# Autodesk Inventor assembly: USE THIS FOR 2018 Practice Drivebase Assembly
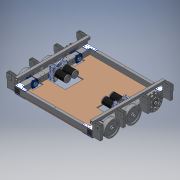
[picture p0: Inventor's stored thumbnail of the model, 180x180]
Saved by Autodesk Inventor 2019 (Build 230136000, 136)
## iProperties
Created: 2018-12-20
Part Number: USE THIS FOR 2018 Practice Drivebase Assembly
Document SubType Name: Assembly
Designer: Tiberus
Sending System: Autodesk Inventor 2018
Preprocessor: ST-DEVELOPER v16.13
Title: C:\Users\maste\OneDrive\Documents\GitHub\2019CAD\USE THIS FOR 2018 Practice Drivebase Assembly.stp
Author: maste
## Documents named in this file (6)
- C:\Users\Tiberus\Documents\Inventor\Robotics\2019CAD-master\2019CAD-master\USE THIS FOR 2018 Practice Drivebase Assembly.iam
- C:\Users\Tiberus\Documents\Inventor\Robotics\2019CAD-master\2019CAD-master\Practice Drivebase Assembly 2018 Version.iam
- C:\Users\Tiberus\Documents\Inventor\Robotics\bumper extrusions.ipt
- C:\Users\Tiberus\Documents\Inventor\Robotics\bumper runner.ipt
- C:\Users\Tiberus\Documents\Inventor\Robotics\bumper attachment.ipt
- C:\Users\Tiberus\Documents\Inventor\Robotics\2019CAD-master\2019CAD-master\USE THIS FOR 2018 Practice Drivebase Assembly\Design Accelerator\Clevis Pin Connection2.iam
## Components (20 placed, 5 different names)
1. Practice Drivebase Assembly 2018 Version:1 [sub-assembly] — Mate:1, Flush:3, Flush:4, Mate:4, Flush:5, Flush:6, Mate:6, Mate:7, Flush:9, Mate:8, Mate:12, Flush:12, Flush:13, Mate:13, Mate:14, Mate:15, Flush:14, Flush:15
2. bumper extrusions:1 — Mate:1, Flush:3, Flush:4, Mate:28, Mate:29, Flush:24
3. bumper extrusions:2 — Mate:8, Mate:30, Flush:25
4. bumper extrusions:3 — Mate:6, Mate:7, Flush:9, Mate:31, Mate:32, Flush:26
5. bumper extrusions:4 — Mate:4, Flush:5, Flush:6, Mate:9, Flush:10, Flush:11, Mate:16, Flush:16, Flush:17
6. bumper extrusions:5 — Mate:15, Flush:14, Flush:15, Mate:17, Mate:24, Flush:23, Mate:25
7. bumper extrusions:6 — Mate:14, Mate:20, Mate:23, Flush:22
8. bumper extrusions:7 — Mate:13, Mate:18, Mate:21, Flush:20
9. bumper extrusions:8 — Mate:12, Flush:12, Flush:13, Flush:18, Flush:19, Mate:19, Flush:21, Mate:22
10. bumper runner:1 — Mate:16, Flush:16, Flush:17
11. bumper attachment:1 — Mate:9, Flush:10, Flush:11
12. bumper runner:2 — Mate:17, Flush:18, Flush:19
13. bumper attachment:2 — Mate:30, Flush:25
14. bumper attachment:3 — Mate:31, Mate:32, Flush:26
15. bumper attachment:4 — Mate:28, Mate:29, Flush:24
16. bumper attachment:5 — Mate:20, Mate:23, Flush:22
17. bumper attachment:6 — Mate:19, Flush:21, Mate:22
18. bumper attachment:7 — Mate:18, Mate:21, Flush:20
19. bumper attachment:8 — Mate:24, Flush:23, Mate:25, Mate:26, Mate:27
20. Clevis Pin Connection:1 [sub-assembly] — Mate:26, Mate:27
## Relationships (49: Mate 27, Flush 22)
- Mate:1: Practice Drivebase Assembly 2018 Version:1 ↔ bumper extrusions:1
- Flush:3: Practice Drivebase Assembly 2018 Version:1 ↔ bumper extrusions:1
- Flush:4: Practice Drivebase Assembly 2018 Version:1 ↔ bumper extrusions:1
- Mate:4: Practice Drivebase Assembly 2018 Version:1 ↔ bumper extrusions:4
- Flush:5: Practice Drivebase Assembly 2018 Version:1 ↔ bumper extrusions:4
- Flush:6: Practice Drivebase Assembly 2018 Version:1 ↔ bumper extrusions:4
- Mate:6: Practice Drivebase Assembly 2018 Version:1 ↔ bumper extrusions:3
- Mate:7: Practice Drivebase Assembly 2018 Version:1 ↔ bumper extrusions:3
- Flush:9: Practice Drivebase Assembly 2018 Version:1 ↔ bumper extrusions:3
- Mate:8: Practice Drivebase Assembly 2018 Version:1 ↔ bumper extrusions:2
- Mate:9: bumper extrusions:4 ↔ bumper attachment:1
- Flush:10: bumper extrusions:4 ↔ bumper attachment:1
- Flush:11: bumper extrusions:4 ↔ bumper attachment:1
- Mate:12: Practice Drivebase Assembly 2018 Version:1 ↔ bumper extrusions:8
- Flush:12: Practice Drivebase Assembly 2018 Version:1 ↔ bumper extrusions:8
- Flush:13: Practice Drivebase Assembly 2018 Version:1 ↔ bumper extrusions:8
- Mate:13: Practice Drivebase Assembly 2018 Version:1 ↔ bumper extrusions:7
- Mate:14: Practice Drivebase Assembly 2018 Version:1 ↔ bumper extrusions:6
- Mate:15: Practice Drivebase Assembly 2018 Version:1 ↔ bumper extrusions:5
- Flush:14: Practice Drivebase Assembly 2018 Version:1 ↔ bumper extrusions:5
- Flush:15: Practice Drivebase Assembly 2018 Version:1 ↔ bumper extrusions:5
- Mate:16: bumper extrusions:4 ↔ bumper runner:1
- Flush:16: bumper extrusions:4 ↔ bumper runner:1
- Flush:17: bumper extrusions:4 ↔ bumper runner:1
- Mate:17: bumper extrusions:5 ↔ bumper runner:2
- Flush:18: bumper extrusions:8 ↔ bumper runner:2
- Flush:19: bumper extrusions:8 ↔ bumper runner:2
- Mate:18: bumper extrusions:7 ↔ bumper attachment:7
- Mate:19: bumper extrusions:8 ↔ bumper attachment:6
- Mate:20: bumper extrusions:6 ↔ bumper attachment:5
- Mate:21: bumper extrusions:7 ↔ bumper attachment:7
- Flush:20: bumper extrusions:7 ↔ bumper attachment:7
- Flush:21: bumper extrusions:8 ↔ bumper attachment:6
- Mate:22: bumper extrusions:8 ↔ bumper attachment:6
- Mate:23: bumper extrusions:6 ↔ bumper attachment:5
- Flush:22: bumper extrusions:6 ↔ bumper attachment:5
- Mate:24: bumper extrusions:5 ↔ bumper attachment:8
- Flush:23: bumper extrusions:5 ↔ bumper attachment:8
- Mate:25: bumper extrusions:5 ↔ bumper attachment:8
- Mate:26: bumper attachment:8 ↔ Clevis Pin Connection:1
- Mate:27: bumper attachment:8 ↔ Clevis Pin Connection:1
- Mate:28: bumper extrusions:1 ↔ bumper attachment:4
- Mate:29: bumper extrusions:1 ↔ bumper attachment:4
- Flush:24: bumper extrusions:1 ↔ bumper attachment:4
- Mate:30: bumper extrusions:2 ↔ bumper attachment:2
- Flush:25: bumper extrusions:2 ↔ bumper attachment:2
- Mate:31: bumper extrusions:3 ↔ bumper attachment:3
- Mate:32: bumper extrusions:3 ↔ bumper attachment:3
- Flush:26: bumper extrusions:3 ↔ bumper attachment:3
